# Autodesk Inventor assembly: HexaDrone
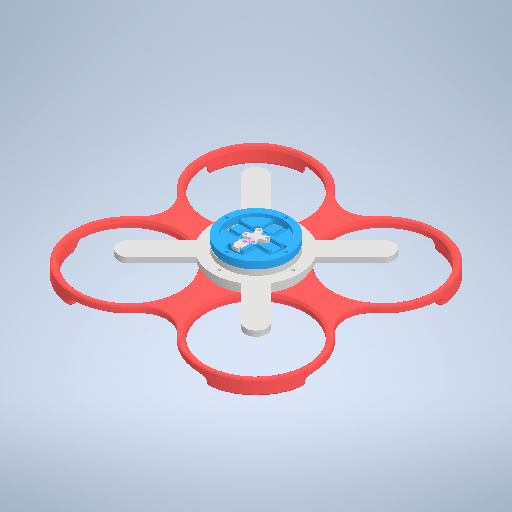
[picture p0: Inventor's stored thumbnail of the model, 512x512]
Saved by Autodesk Inventor 2025.1 (Build 291241020, 241B)
## iProperties
Created: 2024-09-22
Part Number: HexaDrone
Document SubType Name: Assembly
Designer: daare
Author: daare
## Documents named in this file (8)
- C:\Users\SEON06\HexaDrone\HexaDrone.iam
- C:\Users\SEON06\HexaDrone\Base.ipt
- C:\Users\SEON06\HexaDrone\Frame.ipt
- C:\Users\SEON06\HexaDrone\ModuleConnector.ipt
- C:\Users\SEON06\HexaDrone\ModuleConnector_Cap.ipt
- C:\Users\SEON06\HexaDrone\ModuleConnector_Center_Axis.ipt
- C:\Users\SEON06\HexaDrone\ModuleConnector_Outside_Axis.ipt
- C:\Users\SEON06\HexaDrone\ModuleConnector_Axis_Connector.ipt
## Components (7 placed, 7 different names)
1. Base:1 — 메이트:1, 메이트:2, 메이트:3, 메이트:4, 메이트:8, 메이트:11
2. Frame:1 — 메이트:4, 메이트:5, 메이트:6, 메이트:7
3. ModuleConnector_Cap:1 — 메이트:9, 메이트:10, 메이트:12, 메이트:13, 접선:1, 접선:2, 메이트:14, 메이트:15
4. ModuleConnector:1 — 메이트:5, 메이트:6, 메이트:7, 메이트:8, 메이트:9, 메이트:10, 메이트:11, 메이트:12
5. ModuleConnector_Center_Axis:1 — 메이트:13, 접선:1, 접선:2, 메이트:17, 메이트:19
6. ModuleConnector_Outside_Axis:1 — 메이트:14, 메이트:15, 메이트:18
7. ModuleConnector_Axis_Connector:1 — 메이트:17, 메이트:18, 메이트:19
## Relationships (20: Mate 18, Tangent 2)
- 메이트:1 [Mate]: Base:1
- 메이트:2 [Mate]: Base:1
- 메이트:3 [Mate]: Base:1
- 메이트:4 [Mate]: Base:1 ↔ Frame:1
- 메이트:5 [Mate]: Frame:1 ↔ ModuleConnector:1
- 메이트:6 [Mate]: Frame:1 ↔ ModuleConnector:1
- 메이트:7 [Mate]: Frame:1 ↔ ModuleConnector:1
- 메이트:8 [Mate]: Base:1 ↔ ModuleConnector:1
- 메이트:9 [Mate]: ModuleConnector_Cap:1 ↔ ModuleConnector:1
- 메이트:10 [Mate]: ModuleConnector_Cap:1 ↔ ModuleConnector:1
- 메이트:11 [Mate]: Base:1 ↔ ModuleConnector:1
- 메이트:12 [Mate]: ModuleConnector_Cap:1 ↔ ModuleConnector:1
- 메이트:13 [Mate]: ModuleConnector_Cap:1 ↔ ModuleConnector_Center_Axis:1
- 접선:1 [Tangent]: ModuleConnector_Cap:1 ↔ ModuleConnector_Center_Axis:1
- 접선:2 [Tangent]: ModuleConnector_Cap:1 ↔ ModuleConnector_Center_Axis:1
- 메이트:14 [Mate]: ModuleConnector_Cap:1 ↔ ModuleConnector_Outside_Axis:1
- 메이트:15 [Mate]: ModuleConnector_Cap:1 ↔ ModuleConnector_Outside_Axis:1
- 메이트:17 [Mate]: ModuleConnector_Center_Axis:1 ↔ ModuleConnector_Axis_Connector:1
- 메이트:18 [Mate]: ModuleConnector_Outside_Axis:1 ↔ ModuleConnector_Axis_Connector:1
- 메이트:19 [Mate]: ModuleConnector_Center_Axis:1 ↔ ModuleConnector_Axis_Connector:1
